# Autodesk Inventor assembly: Glass Door from Laminated Board For Gluing
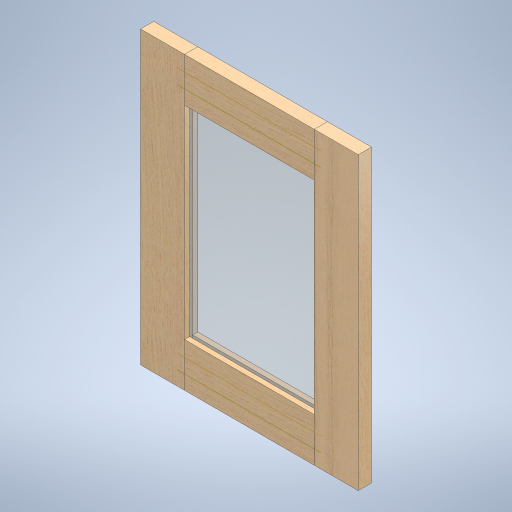
[picture p0: Inventor's stored thumbnail of the model, 512x512]
Saved by Autodesk Inventor 2024 (Build 280153000, 153)
## iProperties
Created: 2017-05-09
Part Number: Glass Door from Laminated Board For Gluing
Document SubType Name: Assembly
Designer: SauliusD
Author: SauliusD
## Documents named in this file (8)
- C:\W4INV 2024 Design\iBOX LIBRARY\Facades\Glass Door from Laminated Board\Glass Door from Laminated Board For Gluing.iam
- C:\W4INV 2024 Design\iBOX LIBRARY\Facades\Glass Door from Laminated Board\Left Frame.ipt
- C:\W4INV 2024 Design\iBOX LIBRARY\Facades\Glass Door from Laminated Board\Top Frame.ipt
- C:\W4INV 2024 Design\iBOX LIBRARY\Facades\Glass Door from Laminated Board\Right Frame.ipt
- C:\W4INV 2024 Design\iBOX LIBRARY\Facades\Glass Door from Laminated Board\Bottom Frame.ipt
- C:\W4INV 2024 Design\iBOX LIBRARY\Facades\Glass Door from Laminated Board\Glass.ipt
- C:\W4INV 2024 Design\_LIBRARY\Fixed joints\Dowel\DOWEL V2\Dowel 8x30 PB T=18.ipt
- C:\W4INV 2023 Design\LIBRARY\Fixed joints\Dowel\DOWEL V2.ipt
## Components (13 placed, 6 different names)
1. Right Frame:1 — Nestled Board Plane:1, Nestled Board Plane:3, Nestled Board Plane:5, Nestled Board Plane:7, Flush:8, Flush:9, Flush:10
2. Top Frame:1 — Flush:1, Flush:2, Pillar Board Plane:1, Pillar Board Plane:2, Pillar Board Plane:3, Pillar Board Plane:4, Pillar Board Plane:5, Pillar Board Plane:6, Pillar Board Plane:7, Pillar Board Plane:8, Flush:5, Flush:6, Flush:7
3. Left Frame:1 — Nestled Board Plane:2, Nestled Board Plane:4, Nestled Board Plane:6, Nestled Board Plane:8
4. Bottom Frame:1 — Flush:3, Flush:4
5. Glass:1
6. Dowel 8x30 PB T=18:1 — Axis Plane:1, Nestled Board Plane:1, Pillar Board Plane:1
7. Dowel 8x30 PB T=18:2 — Axis Plane:2, Nestled Board Plane:2, Pillar Board Plane:2
8. Dowel 8x30 PB T=18:3 — Axis Plane:3, Nestled Board Plane:3, Pillar Board Plane:3
9. Dowel 8x30 PB T=18:4 — Axis Plane:4, Nestled Board Plane:4, Pillar Board Plane:4
10. Dowel 8x30 PB T=18:5 — Axis Plane:5, Nestled Board Plane:5, Pillar Board Plane:5
11. Dowel 8x30 PB T=18:6 — Axis Plane:6, Nestled Board Plane:6, Pillar Board Plane:6
12. Dowel 8x30 PB T=18:7 — Axis Plane:7, Nestled Board Plane:7, Pillar Board Plane:7
13. Dowel 8x30 PB T=18:8 — Axis Plane:8, Nestled Board Plane:8, Pillar Board Plane:8
## Relationships (34: Mate 24, Flush 10)
- Flush:1 (-20 mm): Top Frame:1
- Flush:2 (-20 mm): Top Frame:1
- Flush:3 (-20 mm): Bottom Frame:1
- Flush:4 (-20 mm): Bottom Frame:1
- Axis Plane:1 [Mate]: Dowel 8x30 PB T=18:1
- Nestled Board Plane:1 [Mate]: Right Frame:1 ↔ Dowel 8x30 PB T=18:1
- Pillar Board Plane:1 [Mate] (-9 mm): Top Frame:1 ↔ Dowel 8x30 PB T=18:1
- Axis Plane:2 [Mate]: Dowel 8x30 PB T=18:2
- Nestled Board Plane:2 [Mate]: Left Frame:1 ↔ Dowel 8x30 PB T=18:2
- Pillar Board Plane:2 [Mate] (-9 mm): Top Frame:1 ↔ Dowel 8x30 PB T=18:2
- Axis Plane:3 [Mate]: Dowel 8x30 PB T=18:3
- Nestled Board Plane:3 [Mate]: Right Frame:1 ↔ Dowel 8x30 PB T=18:3
- Pillar Board Plane:3 [Mate] (-9 mm): Top Frame:1 ↔ Dowel 8x30 PB T=18:3
- Axis Plane:4 [Mate]: Dowel 8x30 PB T=18:4
- Nestled Board Plane:4 [Mate]: Left Frame:1 ↔ Dowel 8x30 PB T=18:4
- Pillar Board Plane:4 [Mate] (-9 mm): Top Frame:1 ↔ Dowel 8x30 PB T=18:4
- Axis Plane:5 [Mate]: Dowel 8x30 PB T=18:5
- Nestled Board Plane:5 [Mate]: Right Frame:1 ↔ Dowel 8x30 PB T=18:5
- Pillar Board Plane:5 [Mate] (-9 mm): Top Frame:1 ↔ Dowel 8x30 PB T=18:5
- Axis Plane:6 [Mate]: Dowel 8x30 PB T=18:6
- Nestled Board Plane:6 [Mate]: Left Frame:1 ↔ Dowel 8x30 PB T=18:6
- Pillar Board Plane:6 [Mate] (-9 mm): Top Frame:1 ↔ Dowel 8x30 PB T=18:6
- Axis Plane:7 [Mate]: Dowel 8x30 PB T=18:7
- Nestled Board Plane:7 [Mate]: Right Frame:1 ↔ Dowel 8x30 PB T=18:7
- Pillar Board Plane:7 [Mate] (-9 mm): Top Frame:1 ↔ Dowel 8x30 PB T=18:7
- Axis Plane:8 [Mate]: Dowel 8x30 PB T=18:8
- Nestled Board Plane:8 [Mate]: Left Frame:1 ↔ Dowel 8x30 PB T=18:8
- Pillar Board Plane:8 [Mate] (-9 mm): Top Frame:1 ↔ Dowel 8x30 PB T=18:8
- Flush:5: Top Frame:1
- Flush:6: Top Frame:1
- Flush:7: Top Frame:1
- Flush:8: Right Frame:1
- Flush:9: Right Frame:1
- Flush:10: Right Frame:1
